# Autodesk Inventor assembly: POM_T5_02
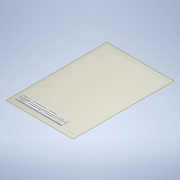
[picture p0: Inventor's stored thumbnail of the model, 180x180]
Saved by Autodesk Inventor 2020 (Build 240168000, 168)
## iProperties
Created: 2021-08-27
Part Number: POM_T5_02
Document SubType Name: Assembly
Designer: Masato
Author: Masato
## Documents named in this file (6)
- C:\Inventor\OpenPlatform_ver3_0\cam\POM_T5_02.iam
- C:\Inventor\OpenPlatform_ver3_0\cam\Disposable_Board.ipt
- C:\Inventor\JIG\Foot_root_block_JIG.ipt
- C:\Inventor\JIG\FrontLink_diagonal_JIG.ipt
- C:\Inventor\JIG\BackLink_diagonal_JIG.ipt
- C:\Inventor\JIG\Leg_joint_yaw_frame_JIG.ipt
## Components (9 placed, 5 different names)
1. Disposable_Board:1 — メイト:2, メイト:1, フラッシュ:1, フラッシュ:2, メイト:4, メイト:5, フラッシュ:3, フラッシュ:4, フラッシュ:5, メイト:7, メイト:8, メイト:9, メイト:10, メイト:11, メイト:12, フラッシュ:6, フラッシュ:7, フラッシュ:8
2. Foot_root_block_JIG:1 — メイト:5, フラッシュ:3, フラッシュ:4, メイト:6, メイト:13
3. Foot_root_block_JIG:2 — メイト:4, メイト:6, フラッシュ:5, メイト:15
4. FrontLink_diagonal_JIG:1 — メイト:7, フラッシュ:6, メイト:13, メイト:14, メイト:16
5. FrontLink_diagonal_JIG:2 — メイト:9, メイト:14, メイト:15, メイト:18
6. BackLink_diagonal_JIG:1 — メイト:10, メイト:17, メイト:18, メイト:21
7. BackLink_diagonal_JIG:2 — メイト:8, フラッシュ:7, メイト:16, メイト:17, メイト:19
8. Leg_joint_yaw_frame_JIG:1 — メイト:12, フラッシュ:8, メイト:19, メイト:20
9. Leg_joint_yaw_frame_JIG:2 — メイト:11, メイト:20, メイト:21
## Relationships (28: Mate 20, Flush 8)
- メイト:2 [Mate]: Disposable_Board:1
- メイト:1 [Mate]: Disposable_Board:1
- フラッシュ:1 [Flush]: Disposable_Board:1
- フラッシュ:2 [Flush]: Disposable_Board:1
- メイト:4 [Mate]: Disposable_Board:1 ↔ Foot_root_block_JIG:2
- メイト:5 [Mate]: Disposable_Board:1 ↔ Foot_root_block_JIG:1
- フラッシュ:3 [Flush] (2.5 mm): Disposable_Board:1 ↔ Foot_root_block_JIG:1
- フラッシュ:4 [Flush] (2.5 mm): Disposable_Board:1 ↔ Foot_root_block_JIG:1
- メイト:6 [Mate] (2.5 mm): Foot_root_block_JIG:1 ↔ Foot_root_block_JIG:2
- フラッシュ:5 [Flush] (2.5 mm): Disposable_Board:1 ↔ Foot_root_block_JIG:2
- メイト:7 [Mate]: Disposable_Board:1 ↔ FrontLink_diagonal_JIG:1
- メイト:8 [Mate]: Disposable_Board:1 ↔ BackLink_diagonal_JIG:2
- メイト:9 [Mate]: Disposable_Board:1 ↔ FrontLink_diagonal_JIG:2
- メイト:10 [Mate]: Disposable_Board:1 ↔ BackLink_diagonal_JIG:1
- メイト:11 [Mate]: Disposable_Board:1 ↔ Leg_joint_yaw_frame_JIG:2
- メイト:12 [Mate]: Disposable_Board:1 ↔ Leg_joint_yaw_frame_JIG:1
- フラッシュ:6 [Flush] (2.5 mm): Disposable_Board:1 ↔ FrontLink_diagonal_JIG:1
- メイト:13 [Mate] (2.5 mm): Foot_root_block_JIG:1 ↔ FrontLink_diagonal_JIG:1
- メイト:14 [Mate] (2.5 mm): FrontLink_diagonal_JIG:1 ↔ FrontLink_diagonal_JIG:2
- メイト:15 [Mate] (2.5 mm): Foot_root_block_JIG:2 ↔ FrontLink_diagonal_JIG:2
- フラッシュ:7 [Flush] (2.5 mm): Disposable_Board:1 ↔ BackLink_diagonal_JIG:2
- メイト:16 [Mate] (2.5 mm): FrontLink_diagonal_JIG:1 ↔ BackLink_diagonal_JIG:2
- メイト:17 [Mate] (2.5 mm): BackLink_diagonal_JIG:1 ↔ BackLink_diagonal_JIG:2
- メイト:18 [Mate] (2.5 mm): FrontLink_diagonal_JIG:2 ↔ BackLink_diagonal_JIG:1
- フラッシュ:8 [Flush] (2.5 mm): Disposable_Board:1 ↔ Leg_joint_yaw_frame_JIG:1
- メイト:19 [Mate] (2.5 mm): BackLink_diagonal_JIG:2 ↔ Leg_joint_yaw_frame_JIG:1
- メイト:20 [Mate] (2.5 mm): Leg_joint_yaw_frame_JIG:1 ↔ Leg_joint_yaw_frame_JIG:2
- メイト:21 [Mate] (2.5 mm): BackLink_diagonal_JIG:1 ↔ Leg_joint_yaw_frame_JIG:2
